# Autodesk Inventor assembly: SingleBoardComputerUnit
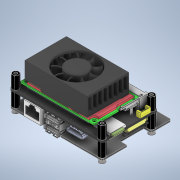
[picture p0: Inventor's stored thumbnail of the model, 180x180]
Saved by Autodesk Inventor 2022.3 (Build 263350000, 350)
## iProperties
Created: 2023-05-14
Part Number: SingleBoardComputerUnit
Document SubType Name: Assembly
Designer: Masato Kubotera
Author: Masato Kubotera
## Documents named in this file (6)
- C:\Users\Masato\Documents\Inventor\Inventor for CIT Brains\SUSTAINA-OP\ElectronicComponents\SingleBoardComputerUnit.iam
- C:\Users\Masato\Documents\Inventor\Inventor for CIT Brains\SUSTAINA-OP\ElectronicComponents\SingleBoardComputer\SingleBoardComputer.ipt
- C:\Users\Masato\Documents\Inventor\Inventor for CIT Brains\SUSTAINA-OP\ElectronicComponents\Board_designed_for_SUSTAINA-OP\A203-V2-Expansion-Board.ipt
- C:\Users\Masato\Documents\Inventor\Inventor for CIT Brains\SUSTAINA-OP\ReadyMade\Spacer\BSL-313BE.ipt
- C:\Users\Masato\Documents\Inventor\Inventor for CIT Brains\SUSTAINA-OP\ReadyMade\Spacer\ASL-312BE.ipt
- C:\Users\Masato\Documents\Inventor\Inventor for CIT Brains\SUSTAINA-OP\ReadyMade\Screw\UC-0306.ipt
## Components (14 placed, 5 different names)
1. SingleBoardComputer:1 — Insert:5, Insert:6, Insert:7, Insert:8, Insert:9, Insert:10, Insert:11, Insert:12
2. A203-V2-Expansion-Board:1 — フラッシュ:1, フラッシュ:2, フラッシュ:3, Insert:1, Insert:2, Insert:3, Insert:4, 挿入:13, 挿入:14, 挿入:15, 挿入:16
3. BSL-313BE:1 — Insert:1, Insert:5
4. BSL-313BE:2 — Insert:2, Insert:6
5. BSL-313BE:3 — Insert:3, Insert:7
6. BSL-313BE:4 — Insert:4, Insert:8
7. ASL-312BE:1 — Insert:9
8. ASL-312BE:2 — Insert:10
9. ASL-312BE:3 — Insert:11
10. ASL-312BE:4 — Insert:12
11. UC-0306:1 — 挿入:13
12. UC-0306:2 — 挿入:14
13. UC-0306:3 — 挿入:15
14. UC-0306:4 — 挿入:16
## Relationships (19: Insert 16, Flush 3)
- フラッシュ:1 [Flush]: A203-V2-Expansion-Board:1
- フラッシュ:2 [Flush]: A203-V2-Expansion-Board:1
- フラッシュ:3 [Flush]: A203-V2-Expansion-Board:1
- Insert:1: A203-V2-Expansion-Board:1 ↔ BSL-313BE:1
- Insert:2: A203-V2-Expansion-Board:1 ↔ BSL-313BE:2
- Insert:3: A203-V2-Expansion-Board:1 ↔ BSL-313BE:3
- Insert:4: A203-V2-Expansion-Board:1 ↔ BSL-313BE:4
- Insert:5: SingleBoardComputer:1 ↔ BSL-313BE:1
- Insert:6: SingleBoardComputer:1 ↔ BSL-313BE:2
- Insert:7: SingleBoardComputer:1 ↔ BSL-313BE:3
- Insert:8: SingleBoardComputer:1 ↔ BSL-313BE:4
- Insert:9: SingleBoardComputer:1 ↔ ASL-312BE:1
- Insert:10: SingleBoardComputer:1 ↔ ASL-312BE:2
- Insert:11: SingleBoardComputer:1 ↔ ASL-312BE:3
- Insert:12: SingleBoardComputer:1 ↔ ASL-312BE:4
- 挿入:13 [Insert]: A203-V2-Expansion-Board:1 ↔ UC-0306:1
- 挿入:14 [Insert]: A203-V2-Expansion-Board:1 ↔ UC-0306:2
- 挿入:15 [Insert]: A203-V2-Expansion-Board:1 ↔ UC-0306:3
- 挿入:16 [Insert]: A203-V2-Expansion-Board:1 ↔ UC-0306:4
